# Autodesk Inventor assembly: Final_Assembly
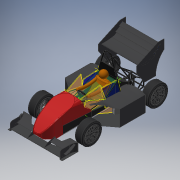
[picture p0: Inventor's stored thumbnail of the model, 180x180]
Saved by Autodesk Inventor 2018.1 (Build 221171000, 171)
## iProperties
Created: 2017-11-02
Part Number: Final_Assembly
Material: 一般
Document SubType Name: Assembly
Designer: kuwano
Author: kuwano
## Documents named in this file (6)
- Z:\各班フォルダ\2018\ボディ\カウル\AeroCAD2018\CAD\Inventor\Final_Assembly.iam
- Z:\各班フォルダ\2018\ボディ\カウル\AeroCAD2018\CAD\Inventor\Assembly(KS-14.ver)\KS-14_SLow\KS-14_SLow_replace.iam
- Z:\各班フォルダ\2018\ボディ\カウル\AeroCAD2018\CAD\Inventor\Aero Parts\R-wing\type6\R-wing.iam
- Z:\各班フォルダ\2018\ボディ\カウル\AeroCAD2018\CAD\Inventor\Aero Parts\Side Pontoon\part\booled.ipt
- Z:\各班フォルダ\2018\ボディ\カウル\AeroCAD2018\CAD\Inventor\Aero Parts\Side Pontoon\part\booled_MIR.ipt
- Z:\各班フォルダ\2018\ボディ\カウル\AeroCAD2018\CAD\Inventor\Aero Parts\F-wing\type7\F-wing.iam
## Components (5 placed, 5 different names)
1. KS-14_SLow_replace:1 [sub-assembly] — メイト:1, メイト:2, メイト:3, メイト:11
2. F-wing:1 [sub-assembly] — フラッシュ:4, メイト:11, 角度:1, フラッシュ:5
3. R-wing:1 [sub-assembly] — フラッシュ:3
4. booled:1 — メイト:5, メイト:6, メイト:7
5. booled_MIR:1 — メイト:8, メイト:9, メイト:10
## Relationships (14: Mate 10, Flush 3, Angle 1)
- メイト:1 [Mate]: KS-14_SLow_replace:1
- メイト:2 [Mate]: KS-14_SLow_replace:1
- メイト:3 [Mate]: KS-14_SLow_replace:1
- フラッシュ:3 [Flush]: R-wing:1
- メイト:5 [Mate]: booled:1
- メイト:6 [Mate]: booled:1
- メイト:7 [Mate]: booled:1
- メイト:8 [Mate]: booled_MIR:1
- メイト:9 [Mate]: booled_MIR:1
- メイト:10 [Mate]: booled_MIR:1
- フラッシュ:4 [Flush]: F-wing:1
- メイト:11 [Mate] (-750 mm): KS-14_SLow_replace:1 ↔ F-wing:1
- 角度:1 [Angle] (0 deg): F-wing:1
- フラッシュ:5 [Flush] (-250 mm): F-wing:1
